# Autodesk Inventor assembly: Carrello semplice
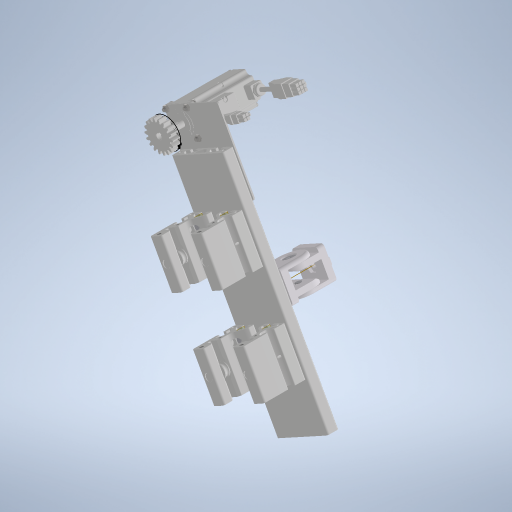
[picture p0: Inventor's stored thumbnail of the model, 512x512]
Saved by Autodesk Inventor 2023 (Build 270158000, 158)
## iProperties
Created: 2021-12-30
Part Number: Carrello semplice
Document SubType Name: Assembly
Designer: matte
Author: matte
## Documents named in this file (14)
- C:\Users\matte\Documents\GitHub\MDM-CyberOrto-CAD\Pezzi singoli\Supporto lineare\Carrello semplice.iam
- C:\Users\matte\Documents\GitHub\MDM-CyberOrto-CAD\Pezzi singoli\Supporto lineare\Piastra-supporto.ipt
- C:\Users\matte\Documents\GitHub\MDM-CyberOrto-CAD\Parker components\08-Linear Application\06-Linear Roller System\01-Roller System 6\30-401.ipt
- C:\Users\matte\Documents\GitHub\MDM-CyberOrto-CAD\Pezzi singoli\Supporto lineare\Doppia Giuntura.iam
- C:\Users\matte\Documents\GitHub\MDM-CyberOrto-CAD\Parker components\05-Handles_Hinges\13-Pivot Joints\23-010.iam
- C:\Users\matte\Documents\GitHub\MDM-CyberOrto-CAD\Parker components\02-Fasteners\10-Standard T-Nuts\20-058.ipt
- C:\Users\matte\Documents\GitHub\MDM-CyberOrto-CAD\Parker components\02-Fasteners\16-Screws\01-Metric Screws\01-Button Head\24-116-8.ipt
- C:\Users\matte\Documents\GitHub\MDM-CyberOrto-CAD\Rack_Pinion\piastra_motore.ipt
- C:\Users\matte\Documents\GitHub\MDM-CyberOrto-CAD\Servo Motor 50W\bch2mba531ca5c.ipt
- C:\Users\matte\Documents\GitHub\MDM-CyberOrto-CAD\Rack_Pinion\Pinion.ipt
- C:\Users\matte\Documents\GitHub\MDM-CyberOrto-CAD\Inventor Support\Content Center Files\it-IT\AS 1474(1)\AS 1474 - M4(1).ipt
- C:\Users\matte\Documents\GitHub\MDM-CyberOrto-CAD\Inventor Support\Content Center Files\it-IT\ISO 1580\ISO 1580 - M4 x 12_.ipt
- C:\Users\matte\Documents\GitHub\MDM-CyberOrto-CAD\Parker components\02-Fasteners\10-Standard T-Nuts\20-050.ipt
- C:\Users\matte\Documents\GitHub\MDM-CyberOrto-CAD\Rack_Pinion\Motor_assembly.iam
## Components (26 placed, 13 different names)
1. Piastra-supporto:1 — Allineato:7, Coincidente:6, Coincidente:7, Coincidente:11, Coincidente:12, Allineato:20, Allineato:21, Angolo:1, Coincidente:21, Coincidente:24, Allineato:26, Coincidente:69, Coincidente:70
2. 30-401:1 — Coincidente:19, Coincidente:56
3. 30-401:2 — Coincidente:24
4. 30-401:3 — Coincidente:68
5. 30-401:4 — Coincidente:8
6. 23-010:1 [sub-assembly] — Allineato:20, Allineato:21, Coincidente:19, Coincidente:20, Coincidente:22, Coincidente:23
7. 20-058:1 — Coincidente:20, Angolo:1, Coincidente:21
8. 24-116-8:1 — Coincidente:22, Coincidente:23
9. 20-050:1 — Coincidente:56
10. 20-050:2 — Coincidente:68
11. Motor_assembly:1 [sub-assembly] — Allineato:26, Coincidente:69, Coincidente:70
12. piastra_motore:1 — Coincidente:27, Allineato:23, Allineato:24, Coincidente:43, Coincidente:44
13. bch2mba531ca5c:1 — Coincidente:27, Allineato:23, Allineato:24, Coincidente:28, Allineato:25, Coincidente:35, Coincidente:36, Coincidente:37, Coincidente:38, Coincidente:39, Coincidente:40, Coincidente:41, Coincidente:42
14. Pinion:1 — Coincidente:28, Allineato:25
15. Doppia Giuntura:2 [sub-assembly] — Coincidente:11, Coincidente:12, Coincidente:15
16. Doppia Giuntura:1 [sub-assembly] — Coincidente:6, Coincidente:7, Coincidente:8, Coincidente:15
17. Doppia Giuntura:3 [sub-assembly]
18. Doppia Giuntura:4 [sub-assembly]
19. AS 1474 - Metrico M4:1 — Coincidente:30
20. ISO 1580 M4 x 12:1 — Coincidente:30, Coincidente:35, Coincidente:36
21. AS 1474 - Metrico M4:2 — Coincidente:43
22. ISO 1580 M4 x 12:2 — Coincidente:37, Coincidente:38
23. AS 1474 - Metrico M4:3
24. ISO 1580 M4 x 12:3 — Coincidente:41, Coincidente:42
25. AS 1474 - Metrico M4:4 — Coincidente:44
26. ISO 1580 M4 x 12:4 — Coincidente:39, Coincidente:40
## Component patterns: (2 elements, first: Doppia Giuntura:2 + Doppia Giuntura:1)
## Relationships (53: Mate 39, Flush 13, Angle 1)
- [Mate]: Piastra-supporto:1 ↔ 30-401:1
- [Flush]: Piastra-supporto:1 ↔ 30-401:1
- [Flush]: Piastra-supporto:1 ↔ 30-401:2
- [Mate]: Piastra-supporto:1 ↔ 30-401:2
- [Mate] (60 mm): 30-401:1 ↔ 30-401:2
- [Mate]: Piastra-supporto:1 ↔ 30-401:3
- [Flush]: Piastra-supporto:1 ↔ 30-401:3
- [Flush]: 30-401:1 ↔ 30-401:3
- [Mate]: Piastra-supporto:1 ↔ 30-401:4
- [Flush]: Piastra-supporto:1 ↔ 30-401:4
- [Flush]: 30-401:2 ↔ 30-401:4
- Allineato:7 [Flush]: Piastra-supporto:1
- Coincidente:6 [Mate]: Piastra-supporto:1 ↔ Doppia Giuntura:1
- Coincidente:7 [Mate]: Piastra-supporto:1 ↔ Doppia Giuntura:1
- Coincidente:8 [Mate]: 30-401:4 ↔ Doppia Giuntura:1
- Coincidente:11 [Mate]: Piastra-supporto:1 ↔ Doppia Giuntura:2
- Coincidente:12 [Mate]: Piastra-supporto:1 ↔ Doppia Giuntura:2
- Coincidente:15 [Mate]: Doppia Giuntura:2 ↔ Doppia Giuntura:1
- Allineato:20 [Flush]: Piastra-supporto:1 ↔ 23-010:1
- Allineato:21 [Flush]: Piastra-supporto:1 ↔ 23-010:1
- Coincidente:19 [Mate] (30 mm): 30-401:1 ↔ 23-010:1
- Coincidente:20 [Mate]: 23-010:1 ↔ 20-058:1
- Angolo:1 [Angle] (0 deg): Piastra-supporto:1 ↔ 20-058:1
- Coincidente:21 [Mate]: Piastra-supporto:1 ↔ 20-058:1
- Coincidente:22 [Mate]: 23-010:1 ↔ 24-116-8:1
- Coincidente:23 [Mate]: 23-010:1 ↔ 24-116-8:1
- Coincidente:24 [Mate] (60 mm): Piastra-supporto:1 ↔ 30-401:2
- Coincidente:27 [Mate]: piastra_motore:1 ↔ bch2mba531ca5c:1
- Allineato:23 [Flush]: piastra_motore:1 ↔ bch2mba531ca5c:1
- Allineato:24 [Flush]: piastra_motore:1 ↔ bch2mba531ca5c:1
- Coincidente:28 [Mate]: bch2mba531ca5c:1 ↔ Pinion:1
- Allineato:25 [Flush] (-10 mm): bch2mba531ca5c:1 ↔ Pinion:1
- [Mate]: AS 1474 - Metrico M4:1 ↔ ISO 1580 M4 x 12:1
- Coincidente:30 [Mate] (7.715 mm): AS 1474 - Metrico M4:1 ↔ ISO 1580 M4 x 12:1
- [Mate]: AS 1474 - Metrico M4:2 ↔ ISO 1580 M4 x 12:2
- [Mate]: AS 1474 - Metrico M4:3 ↔ ISO 1580 M4 x 12:3
- [Mate] (7.715 mm): AS 1474 - Metrico M4:3 ↔ ISO 1580 M4 x 12:3
- [Mate]: AS 1474 - Metrico M4:4 ↔ ISO 1580 M4 x 12:4
- Coincidente:35 [Mate]: bch2mba531ca5c:1 ↔ ISO 1580 M4 x 12:1
- Coincidente:36 [Mate]: bch2mba531ca5c:1 ↔ ISO 1580 M4 x 12:1
- Coincidente:37 [Mate]: bch2mba531ca5c:1 ↔ ISO 1580 M4 x 12:2
- Coincidente:38 [Mate]: bch2mba531ca5c:1 ↔ ISO 1580 M4 x 12:2
- Coincidente:39 [Mate]: bch2mba531ca5c:1 ↔ ISO 1580 M4 x 12:4
- Coincidente:40 [Mate]: bch2mba531ca5c:1 ↔ ISO 1580 M4 x 12:4
- Coincidente:41 [Mate]: bch2mba531ca5c:1 ↔ ISO 1580 M4 x 12:3
- Coincidente:42 [Mate]: bch2mba531ca5c:1 ↔ ISO 1580 M4 x 12:3
- Coincidente:43 [Mate]: piastra_motore:1 ↔ AS 1474 - Metrico M4:2
- Coincidente:44 [Mate]: piastra_motore:1 ↔ AS 1474 - Metrico M4:4
- Coincidente:56 [Mate]: 30-401:1 ↔ 20-050:1
- Coincidente:68 [Mate]: 30-401:3 ↔ 20-050:2
- Allineato:26 [Flush]: Piastra-supporto:1 ↔ Motor_assembly:1
- Coincidente:69 [Mate]: Piastra-supporto:1 ↔ Motor_assembly:1
- Coincidente:70 [Mate] (10 mm): Piastra-supporto:1 ↔ Motor_assembly:1
## Named parameters: d78_d351 = 0 mm, d79_d351 = 0 mm, d80_d77 = 7.715 mm, d81_d78_d351 = 0 mm
